# Autodesk Inventor assembly: V2-Output-CIM
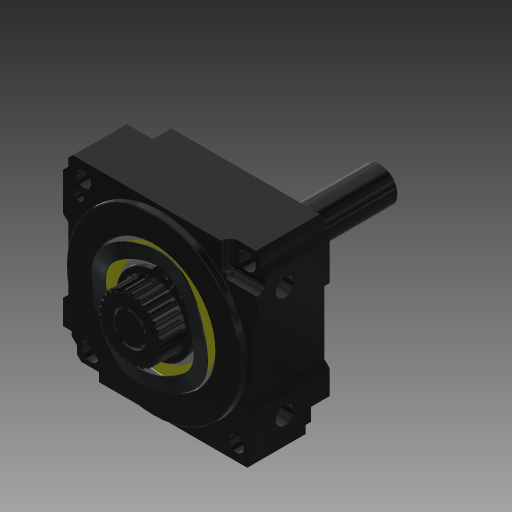
[picture p0: Inventor's stored thumbnail of the model, 512x512]
Saved by Autodesk Inventor 2023 (Build 270158000, 158)
## iProperties
Created: 2018-08-19
Part Number: V2-Output-CIM
Document SubType Name: Assembly
Mass: 68.0389 g
Surface Area: 377.272 cm^2
Volume: 60.8381 cm^3
Density: 1.11836 g/cm^3
## Documents named in this file (8)
- C:\Users\Cal\Desktop\Robotics\Design\Collaborative\Collaborative Parts Library\General Gearboxes\Planetaries\Versaplanetary\V2 Stages\V2 Output Stage\VP V2 Output Stage CIM.iam
- C:\Users\Cal\Desktop\Robotics\Design\Collaborative\Collaborative Parts Library\General Gearboxes\Planetaries\Versaplanetary\V2 Stages\V2 Output Housing.ipt
- C:\Users\Cal\Desktop\Robotics\Design\Collaborative\Collaborative Parts Library\General Gearboxes\Planetaries\Versaplanetary\V2 Stages\Wave Washer.ipt
- C:\Users\Cal\Desktop\Robotics\Design\Collaborative\Collaborative Parts Library\General Gearboxes\Planetaries\Versaplanetary\V2 Stages\Retaining Ring.ipt
- C:\Users\Cal\Desktop\Robotics\Design\Collaborative\Collaborative Parts Library\General Gearboxes\Planetaries\Versaplanetary\Output Shafts\VP CIM Output.ipt
- C:\Users\Cal\Desktop\Robotics\Design\Collaborative\Collaborative Parts Library\Power Transfer\Bearings and Bushings\Bearings\6902ZZ.ipt
- E:\Elipse 6814\Elipse Parts Library\Shaft Accessories\Bearings.ipt
- C:\Users\Cal\Desktop\Robotics\Design\Collaborative\Collaborative Parts Library\General Gearboxes\Planetaries\Versaplanetary\V2 Stages\V2 Output Stage.iam
## Components (6 placed, 5 different names)
1. V2 Output Housing:1 — Insert:2, Mate:2, Insert:18, Mate:3, Angle:6, Flush:7
2. 6902ZZ:1 — Insert:2, Insert:23
3. 6902ZZ:2 — Insert:18, Insert:24
4. Wave Washer:1 — Mate:2
5. Retaining Ring:1 — Angle:4, Insert:23
6. VP CIM Output:1 — Angle:4, Insert:24
## Relationships (9: Insert 4, Mate 2, Angle 2, Flush 1)
- Insert:2: V2 Output Housing:1 ↔ 6902ZZ:1
- Mate:2: V2 Output Housing:1 ↔ Wave Washer:1
- Angle:4 (0 deg): Retaining Ring:1 ↔ VP CIM Output:1
- Insert:18: V2 Output Housing:1 ↔ 6902ZZ:2
- Insert:23 (0.508 mm): 6902ZZ:1 ↔ Retaining Ring:1
- Insert:24: 6902ZZ:2 ↔ VP CIM Output:1
- Mate:3: V2 Output Housing:1
- Angle:6 (0 deg): V2 Output Housing:1
- Flush:7: V2 Output Housing:1
